# Autodesk Inventor assembly: Carriage_Assembly
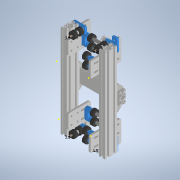
[picture p0: Inventor's stored thumbnail of the model, 180x180]
Saved by Autodesk Inventor 2021 (Build 250183000, 183)
## iProperties
Created: 2021-09-08
Part Number: Carriage_Assembly
Document SubType Name: Assembly
Designer: Jorian Brusind
Author: Jorian Brusind
## Documents named in this file (11)
- C:\Users\Jorian Brusind\Documents\GitHub\PersonalProjects\HyperRail\Inventor Files\Carriage_Assembly.iam
- C:\Users\Jorian Brusind\Documents\GitHub\PersonalProjects\Inventor Projects\Useful models\8020_Sets\IPT_20_Series\IPT_20_Series\20-2040_150mm.ipt
- C:\Users\Jorian Brusind\Documents\GitHub\PersonalProjects\HyperRail\Inventor Files\X_CarriageL_V2_0_Short.iam
- C:\Users\Jorian Brusind\Documents\GitHub\PersonalProjects\HyperRail\Inventor Files\X_CarriageR_V2_0_Short.iam
- C:\Users\Jorian Brusind\Documents\GitHub\PersonalProjects\HyperRail\Inventor Files\X_CarriageR_V2_0.iam
- C:\Users\Jorian Brusind\Documents\GitHub\PersonalProjects\HyperRail\Inventor Files\X_Carriage_V2_0.iam
- C:\Users\Jorian Brusind\Documents\GitHub\PersonalProjects\Inventor Projects\Useful models\8020_Sets\IPT_20_Series\Extra_20_Series\8020_14056m\14056_m.ipt
- C:\Users\Jorian Brusind\Documents\GitHub\PersonalProjects\HyperRail\Inventor Files\Buffer.iam
- C:\Users\Jorian Brusind\Documents\GitHub\PersonalProjects\Inventor Projects\Useful models\Metric Spacer_Standoffs\hex spacer standoff nut M5 L30.ipt
- C:\Users\Jorian Brusind\Documents\GitHub\PersonalProjects\HyperRail\Inventor Files\Carriage_Horizontal_Spacer.ipt
- C:\Users\Jorian Brusind\Documents\GitHub\PersonalProjects\Inventor Projects\Useful models\8020_Sets\IPT_20_Series\IPT_20_Series\20-2040_400mm.ipt
## Components (21 placed, 10 different names)
1. 20-2040_150mm:1 — Mate:20, Mate:21, Mate:22, Mate:23, Mate:80, Flush:33
2. X_CarriageL_V2_0_Short:1 [sub-assembly] — Mate:97, Flush:48, Flush:49, Flush:50, Flush:51, Mate:99, Mate:102
3. X_CarriageR_V2_0_Short:1 [sub-assembly] — Mate:89, Mate:90, Flush:44, Flush:45, Flush:46, Mate:92, Mate:93, Mate:95, Mate:104
4. X_CarriageR_V2_0:1 [sub-assembly] — Mate:96, Flush:50, Flush:51, Mate:100, Mate:101, Mate:103, Flush:56
5. 14056_m:1 — Mate:21, Flush:26, Flush:38
6. 14056_m:2 — Mate:20, Flush:25, Flush:26, Mate:70, Flush:37, Flush:39, Mate:105
7. 14056_m:3 — Mate:22, Flush:13
8. 14056_m:4 — Mate:23, Flush:13, Flush:28, Mate:72
9. Buffer:1 [sub-assembly] — Mate:82, Flush:41, Flush:54
10. Buffer:2 [sub-assembly] — Mate:86, Mate:90, Flush:47, Flush:55
11. Buffer:3 [sub-assembly] — Flush:42, Mate:87, Flush:43
12. Buffer:4 [sub-assembly] — Mate:88, Flush:49, Flush:52, Flush:53
13. hex spacer standoff nut M5 L30:2 — Mate:95, Mate:98, Mate:104
14. hex spacer standoff nut M5 L30:3 — Mate:93, Mate:94
15. hex spacer standoff nut M5 L30:4 — Mate:99, Mate:100, Mate:101
16. hex spacer standoff nut M5 L30:6 — Mate:102, Mate:103
17. Carriage_Horizontal_Spacer:1 — Flush:28, Mate:72, Mate:79, Mate:80
18. Carriage_Horizontal_Spacer:2 — Flush:25, Mate:70, Mate:84, Flush:37, Flush:38
19. 20-2040_400mm:1 — Flush:30, Mate:75, Mate:76, Mate:79, Flush:33, Flush:36, Mate:86, Mate:88, Mate:89, Flush:44, Flush:47, Mate:97, Flush:48, Flush:52, Flush:53, Flush:55
20. 20-2040_400mm:2 — Flush:30, Flush:36, Mate:82, Mate:84, Flush:39, Flush:41, Flush:42, Mate:87, Flush:43, Mate:91, Mate:96, Flush:54
21. X_Carriage_V2_0:1 [sub-assembly] — Mate:91, Flush:45, Flush:46, Mate:92, Mate:94, Mate:98, Mate:105, Flush:56
## Relationships (58: Mate 32, Flush 26)
- Mate:20: 20-2040_150mm:1 ↔ 14056_m:2
- Mate:21: 20-2040_150mm:1 ↔ 14056_m:1
- Mate:22: 20-2040_150mm:1 ↔ 14056_m:3
- Mate:23: 20-2040_150mm:1 ↔ 14056_m:4
- Flush:13: 14056_m:3 ↔ 14056_m:4
- Flush:25: 14056_m:2 ↔ Carriage_Horizontal_Spacer:2
- Flush:26: 14056_m:1 ↔ 14056_m:2
- Mate:70: 14056_m:2 ↔ Carriage_Horizontal_Spacer:2
- Flush:28: 14056_m:4 ↔ Carriage_Horizontal_Spacer:1
- Mate:72: 14056_m:4 ↔ Carriage_Horizontal_Spacer:1
- Flush:30: 20-2040_400mm:1 ↔ 20-2040_400mm:2
- Mate:75: 20-2040_400mm:1
- Mate:76: 20-2040_400mm:1
- Mate:79: Carriage_Horizontal_Spacer:1 ↔ 20-2040_400mm:1
- Mate:80: 20-2040_150mm:1 ↔ Carriage_Horizontal_Spacer:1
- Flush:33: 20-2040_150mm:1 ↔ 20-2040_400mm:1
- Flush:36: 20-2040_400mm:1 ↔ 20-2040_400mm:2
- Mate:82: Buffer:1 ↔ 20-2040_400mm:2
- Mate:84: Carriage_Horizontal_Spacer:2 ↔ 20-2040_400mm:2
- Flush:37: 14056_m:2 ↔ Carriage_Horizontal_Spacer:2
- Flush:38: 14056_m:1 ↔ Carriage_Horizontal_Spacer:2
- Flush:39: 14056_m:2 ↔ 20-2040_400mm:2
- Mate:86: Buffer:2 ↔ 20-2040_400mm:1
- Flush:41: Buffer:1 ↔ 20-2040_400mm:2
- Flush:42: Buffer:3 ↔ 20-2040_400mm:2
- Mate:87: Buffer:3 ↔ 20-2040_400mm:2
- Flush:43: Buffer:3 ↔ 20-2040_400mm:2
- Mate:88: Buffer:4 ↔ 20-2040_400mm:1
- Mate:89: X_CarriageR_V2_0_Short:1 ↔ 20-2040_400mm:1
- Mate:90: X_CarriageR_V2_0_Short:1 ↔ Buffer:2
- Flush:44: X_CarriageR_V2_0_Short:1 ↔ 20-2040_400mm:1
- Mate:91: 20-2040_400mm:2 ↔ X_Carriage_V2_0:1
- Flush:45: X_CarriageR_V2_0_Short:1 ↔ X_Carriage_V2_0:1
- Flush:46: X_CarriageR_V2_0_Short:1 ↔ X_Carriage_V2_0:1
- Mate:92: X_CarriageR_V2_0_Short:1 ↔ X_Carriage_V2_0:1
- Mate:93: X_CarriageR_V2_0_Short:1 ↔ hex spacer standoff nut M5 L30:3
- Mate:94: hex spacer standoff nut M5 L30:3 ↔ X_Carriage_V2_0:1
- Mate:95: X_CarriageR_V2_0_Short:1 ↔ hex spacer standoff nut M5 L30:2
- Flush:47: Buffer:2 ↔ 20-2040_400mm:1
- Mate:96: X_CarriageR_V2_0:1 ↔ 20-2040_400mm:2
- Mate:97: X_CarriageL_V2_0_Short:1 ↔ 20-2040_400mm:1
- Flush:48: X_CarriageL_V2_0_Short:1 ↔ 20-2040_400mm:1
- Flush:49: X_CarriageL_V2_0_Short:1 ↔ Buffer:4
- Flush:50: X_CarriageL_V2_0_Short:1 ↔ X_CarriageR_V2_0:1
- Flush:51: X_CarriageL_V2_0_Short:1 ↔ X_CarriageR_V2_0:1
- Mate:98: hex spacer standoff nut M5 L30:2 ↔ X_Carriage_V2_0:1
- Mate:99: X_CarriageL_V2_0_Short:1 ↔ hex spacer standoff nut M5 L30:4
- Mate:100: X_CarriageR_V2_0:1 ↔ hex spacer standoff nut M5 L30:4
- Mate:101: X_CarriageR_V2_0:1 ↔ hex spacer standoff nut M5 L30:4
- Mate:102: X_CarriageL_V2_0_Short:1 ↔ hex spacer standoff nut M5 L30:6
- Mate:103: X_CarriageR_V2_0:1 ↔ hex spacer standoff nut M5 L30:6
- Mate:104: X_CarriageR_V2_0_Short:1 ↔ hex spacer standoff nut M5 L30:2
- Flush:52: Buffer:4 ↔ 20-2040_400mm:1
- Flush:53: Buffer:4 ↔ 20-2040_400mm:1
- Flush:54: Buffer:1 ↔ 20-2040_400mm:2
- Flush:55: Buffer:2 ↔ 20-2040_400mm:1
- Mate:105 (40 mm): 14056_m:2 ↔ X_Carriage_V2_0:1
- Flush:56: X_CarriageR_V2_0:1 ↔ X_Carriage_V2_0:1
